# Autodesk Inventor assembly: chess-set-one
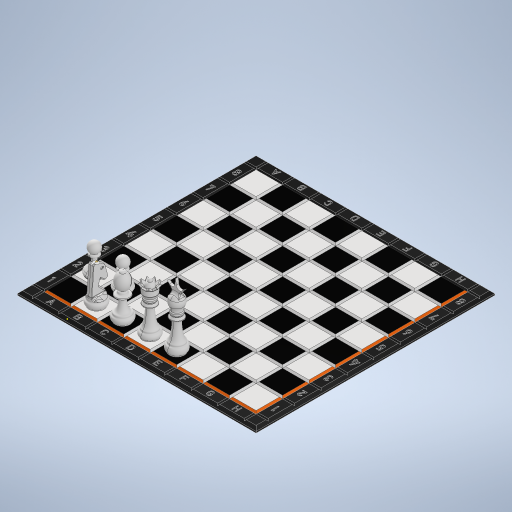
[picture p0: Inventor's stored thumbnail of the model, 512x512]
Saved by Autodesk Inventor 2024.1 (Build 281209000, 209)
## iProperties
Created: 2025-07-31
Part Number: chess-set-one
Document SubType Name: Assembly
Designer: iwheard
Author: iwheard
## Documents named in this file (7)
- C:\Users\iwheard\Documents\0004-CAD\3D-cad-main\chess-set\chess-set-one.iam
- C:\Users\iwheard\Documents\0004-CAD\3D-cad-main\chess-set\board.ipt
- C:\Users\iwheard\Documents\0004-CAD\3D-cad-main\chess-set\pawn-white-v2.ipt
- C:\Users\iwheard\Documents\0004-CAD\3D-cad-main\chess-set\queen-white.ipt
- C:\Users\iwheard\Documents\0004-CAD\3D-cad-main\chess-set\king-white.ipt
- C:\Users\iwheard\Documents\0004-CAD\3D-cad-main\chess-set\bishop-white.ipt
- C:\Users\iwheard\Documents\0004-CAD\3D-cad-main\chess-set\knight-white.ipt
## Components (7 placed, 6 different names)
1. board:1 — Mate:1, Angle:1
2. pawn-white-v2:1 — Mate:1, Angle:1
3. pawn-white-v2:2
4. queen-white:1
5. king-white:1
6. bishop-white:1
7. knight-white:1
## Relationships (2: Mate 1, Angle 1)
- Mate:1: board:1 ↔ pawn-white-v2:1
- Angle:1 (0 deg): board:1 ↔ pawn-white-v2:1
